# Autodesk Inventor assembly: Assembly_for_print
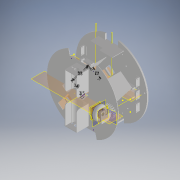
[picture p0: Inventor's stored thumbnail of the model, 180x180]
Saved by Autodesk Inventor 2020 (Build 240168000, 168)
## iProperties
Created: 2020-10-03
Part Number: Assembly_for_print
Document SubType Name: Assembly
Designer: Sičaja
Author: Sičaja
## Documents named in this file (7)
- C:\Users\Sicaja\Fakultet elektrotehnike, strojarstva i brodogradnje\Mirko Pezo - Rescue Maze Robot\Strojarstvo\Inverntor_parts_for_print\Assembly_for_print.iam
- C:\Users\Sicaja\Fakultet elektrotehnike, strojarstva i brodogradnje\Mirko Pezo - Rescue Maze Robot\Strojarstvo\Inverntor_parts_for_print\DropMechanism_v.2.0.ipt
- C:\Users\Sicaja\Fakultet elektrotehnike, strojarstva i brodogradnje\Mirko Pezo - Rescue Maze Robot\Strojarstvo\Inverntor_parts_for_print\KonstrukcijaDonjiDio_v.1.1.ipt
- C:\Users\Sicaja\Documents\Projects\3D Drawings\Inventor_draws\Robocup\Inverntor_parts_for_print\Gornja_konstrukcija_s_držačima_assembly_converted_v.3.0.ipt
- C:\Users\Sicaja\Fakultet elektrotehnike, strojarstva i brodogradnje\Mirko Pezo - Rescue Maze Robot\Strojarstvo\Inverntor_parts_for_print\DrzacZaPrednjiKotač_v.1.0.ipt
- C:\Users\Sicaja\Fakultet elektrotehnike, strojarstva i brodogradnje\Mirko Pezo - Rescue Maze Robot\Strojarstvo\Inverntor_parts_for_print\PrednjiKotač_635z_lezaj_v.2.0.ipt
- C:\Users\Sicaja\Documents\Projects\3D Drawings\Inventor_draws\Robocup\Inverntor_parts_for_print\AdfruitThermalSensor\Camara AMG8833.ipt
## Components (6 placed, 6 different names)
1. DropMechanism_v.2.0:1 — Mate:1, Mate:2, Flush:1
2. KonstrukcijaDonjiDio_v.1.1:1 — Mate:1, Mate:2, Flush:1, Mate:3, Mate:4, Mate:14, Insert:3, Mate:15, Insert:5, Insert:6
3. Gornja_konstrukcija_s_držačima_assembly_converted_v.3.0:1 — Mate:3, Mate:4, Mate:15, Insert:5, Insert:6, Mate:16, Flush:2, Flush:3
4. DrzacZaPrednjiKotač_v.1.0:1 — Mate:14, Insert:3, Insert:4
5. PrednjiKotač_635z_lezaj_v.2.0:1 — Insert:4
6. Camara AMG8833:1 — Mate:16, Flush:2, Flush:3
## Relationships (14: Mate 7, Insert 4, Flush 3)
- Mate:1: DropMechanism_v.2.0:1 ↔ KonstrukcijaDonjiDio_v.1.1:1
- Mate:2 (6 mm): DropMechanism_v.2.0:1 ↔ KonstrukcijaDonjiDio_v.1.1:1
- Flush:1 (-12 mm): DropMechanism_v.2.0:1 ↔ KonstrukcijaDonjiDio_v.1.1:1
- Mate:3 (60 mm): KonstrukcijaDonjiDio_v.1.1:1 ↔ Gornja_konstrukcija_s_držačima_assembly_converted_v.3.0:1
- Mate:4: KonstrukcijaDonjiDio_v.1.1:1 ↔ Gornja_konstrukcija_s_držačima_assembly_converted_v.3.0:1
- Mate:14: KonstrukcijaDonjiDio_v.1.1:1 ↔ DrzacZaPrednjiKotač_v.1.0:1
- Insert:3: KonstrukcijaDonjiDio_v.1.1:1 ↔ DrzacZaPrednjiKotač_v.1.0:1
- Insert:4: DrzacZaPrednjiKotač_v.1.0:1 ↔ PrednjiKotač_635z_lezaj_v.2.0:1
- Mate:15 (60 mm): KonstrukcijaDonjiDio_v.1.1:1 ↔ Gornja_konstrukcija_s_držačima_assembly_converted_v.3.0:1
- Insert:5: KonstrukcijaDonjiDio_v.1.1:1 ↔ Gornja_konstrukcija_s_držačima_assembly_converted_v.3.0:1
- Insert:6: KonstrukcijaDonjiDio_v.1.1:1 ↔ Gornja_konstrukcija_s_držačima_assembly_converted_v.3.0:1
- Mate:16: Gornja_konstrukcija_s_držačima_assembly_converted_v.3.0:1 ↔ Camara AMG8833:1
- Flush:2 (0.95 mm): Gornja_konstrukcija_s_držačima_assembly_converted_v.3.0:1 ↔ Camara AMG8833:1
- Flush:3: Gornja_konstrukcija_s_držačima_assembly_converted_v.3.0:1 ↔ Camara AMG8833:1
